# Autodesk Inventor assembly: RUKA ROBOT ASSEMBLY
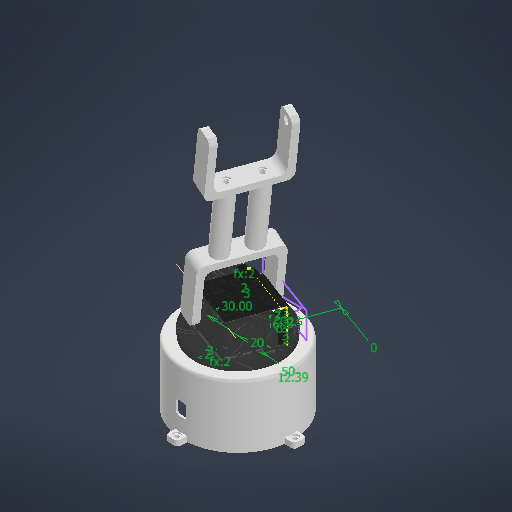
[picture p0: Inventor's stored thumbnail of the model, 512x512]
Saved by Autodesk Inventor 2026 (Build 300175000, 175)
## iProperties
Created: 2025-04-11
Part Number: RUKA ROBOT ASSEMBLY
Document SubType Name: Assembly
Designer: janpa
Author: janpa
## Documents named in this file (6)
- C:\Users\janpa\OneDrive\Plocha\Hackaton\Hackathon25\3d\RUKA ROBOT ASSEMBLY.iam
- C:\Users\janpa\Downloads\MG995-Servo.ipt
- C:\Users\janpa\OneDrive\Plocha\Hackaton\Hackathon25\3d\ruka base.ipt
- C:\Users\janpa\OneDrive\Plocha\Hackaton\Hackathon25\3d\rotacniZaklad.ipt
- C:\Users\janpa\OneDrive\Plocha\Hackaton\Hackathon25\3d\ruka_part spodni.ipt
- C:\Users\janpa\OneDrive\Plocha\Hackaton\Hackathon25\3d\extendo1.ipt
## Components (8 placed, 5 different names)
1. MG995-Servo:1 — Mate:1, Mate:2, Mate:4
2. ruka base:1 — Mate:1, Mate:5
3. rotacniZaklad:1 — Mate:2, Mate:4, Mate:5, Mate:6, Mate:7, Mate:8
4. MG995-Servo:2 — Mate:6, Mate:7, Mate:8, Mate:9, Mate:10
5. ruka_part spodni:1 — Mate:9, Mate:10, Mate:11, Mate:12, Mate:13, Mate:14
6. extendo1:1 — Mate:11, Mate:12, Mate:16, Mate:17
7. extendo1:2 — Mate:13, Mate:14, Mate:15, Mate:18
8. ruka_part spodni:2 — Mate:15, Mate:16, Mate:17, Mate:18
## Relationships (17: Mate 17)
- Mate:1: MG995-Servo:1 ↔ ruka base:1
- Mate:2: MG995-Servo:1 ↔ rotacniZaklad:1
- Mate:4: MG995-Servo:1 ↔ rotacniZaklad:1
- Mate:5: ruka base:1 ↔ rotacniZaklad:1
- Mate:6: rotacniZaklad:1 ↔ MG995-Servo:2
- Mate:7: rotacniZaklad:1 ↔ MG995-Servo:2
- Mate:8: rotacniZaklad:1 ↔ MG995-Servo:2
- Mate:9: MG995-Servo:2 ↔ ruka_part spodni:1
- Mate:10: MG995-Servo:2 ↔ ruka_part spodni:1
- Mate:11: ruka_part spodni:1 ↔ extendo1:1
- Mate:12: ruka_part spodni:1 ↔ extendo1:1
- Mate:13: ruka_part spodni:1 ↔ extendo1:2
- Mate:14: ruka_part spodni:1 ↔ extendo1:2
- Mate:15: extendo1:2 ↔ ruka_part spodni:2
- Mate:16: extendo1:1 ↔ ruka_part spodni:2
- Mate:17: extendo1:1 ↔ ruka_part spodni:2
- Mate:18: extendo1:2 ↔ ruka_part spodni:2
